# Autodesk Inventor assembly: Frame
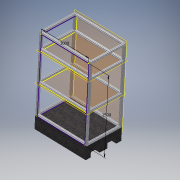
[picture p0: Inventor's stored thumbnail of the model, 180x180]
Saved by Autodesk Inventor 2016 (Build 200138000, 138)
## iProperties
Created: 2015-07-26
Part Number: Frame
Document SubType Name: Assembly
Designer: myhome
Mass: 435549 g
Surface Area: 93513.9 cm^2
Volume: 178817 cm^3
Density: 2.43572 g/cm^3
_SolveAssemblyDoc: Frame Generator Solve Assembly
_Version: 15.0.0
Author: myhome
## Documents named in this file (4)
- C:\Users\myhome\Documents\Inventor\Printer\Frame.iam
- C:\Users\myhome\Documents\Inventor\Printer\Part1.ipt
- C:\Users\myhome\Documents\Inventor\Printer\Frame\Frame\Frame0001.iam
- C:\Users\myhome\Documents\Inventor\Printer\EpoxyGraniteBase\GraniteEpoxyBase.ipt
## Components (3 placed, 3 different names)
1. FrameSkeleton
2. Frame0001:1 [sub-assembly] — Rigid:1
3. GraniteEpoxyBase:1 — Rigid:1
## Relationships (1: WeldJoint 1)
- Rigid:1 [WeldJoint]: Frame0001:1 ↔ GraniteEpoxyBase:1
